# Autodesk Inventor assembly: Baugruppe
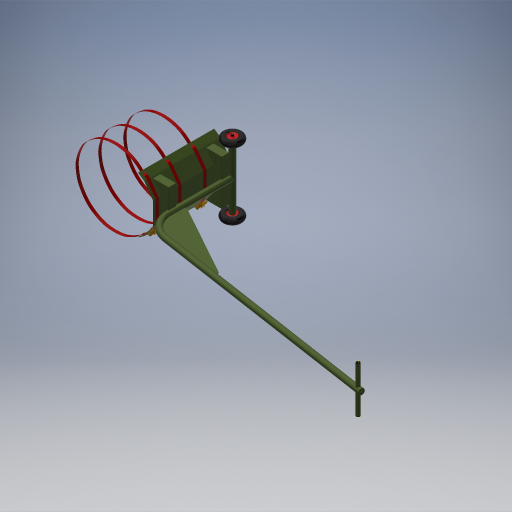
[picture p0: Inventor's stored thumbnail of the model, 512x512]
Saved by Autodesk Inventor 2023.2 (Build 272271000, 271)
## iProperties
Created: 2023-02-05
Part Number: Baugruppe
Material: Generisch
Document SubType Name: Assembly
Designer: Raoul Messerli
Author: Raoul Messerli
## Documents named in this file (8)
- E:\GitHub\Pflanzenwagen\40_Realisieren\20_Inventor\40_Baugruppen\Baugruppe.iam
- E:\GitHub\Pflanzenwagen\40_Realisieren\20_Inventor\40_Baugruppen\Schweiss Baugruppe.iam
- E:\GitHub\Pflanzenwagen\40_Realisieren\20_Inventor\20_Einkaufteile\Wheel.ipt
- E:\GitHub\Pflanzenwagen\40_Realisieren\20_Inventor\20_Einkaufteile\BN 161 1118811 prevailing torque type hex lock nut M20_Steel 6.ipt
- E:\GitHub\Pflanzenwagen\40_Realisieren\20_Inventor\20_Einkaufteile\Round_sliders.ipt
- E:\GitHub\Pflanzenwagen\40_Realisieren\20_Inventor\20_Einkaufteile\RatchetStrap\Strap for Pflanzenwagen.ipt
- E:\GitHub\Pflanzenwagen\40_Realisieren\20_Inventor\20_Einkaufteile\Gummi Matte.ipt
- E:\GitHub\Pflanzenwagen\40_Realisieren\20_Inventor\20_Einkaufteile\RatchetStrap\RatchetStrap\RatchetStrap.iam
## Components (14 placed, 7 different names)
1. Schweiss Baugruppe:1 [sub-assembly] — Fluchtend:1, Fluchtend:2, Fluchtend:3, Passend:1, Passend:2, Passend:3, Passend:4, Passend:5, Passend:7, Passend:9, Passend:10, Passend:11, Passend:12, Passend:14, Passend:18, Passend:21, Passend:22, Fluchtend:4, Passend:24, Passend:26, Passend:27
2. Wheel:1 — Passend:1, Passend:3, Passend:6
3. Wheel:2 — Passend:2, Passend:4, Passend:8
4. BN 161 1118811 prevailing torque type hex lock nut M20_Steel 6:1 — Passend:5, Passend:6
5. BN 161 1118811 prevailing torque type hex lock nut M20_Steel 6:2 — Passend:7, Passend:8
6. Round_sliders:1 — Passend:9, Passend:10
7. Round_sliders:2 — Passend:11, Passend:12
8. Strap for Pflanzenwagen:1 — Passend:13, Passend:14, Passend:15, Passend:29
9. Strap for Pflanzenwagen:2 — Passend:16, Passend:17, Passend:18, Passend:28
10. Strap for Pflanzenwagen:3 — Passend:19, Passend:20, Passend:21, Passend:25
11. Gummi Matte:1 — Passend:22, Fluchtend:4, Passend:23
12. RatchetStrap:1 [sub-assembly] — Passend:24, Passend:25
13. RatchetStrap:2 [sub-assembly] — Passend:26, Passend:28
14. RatchetStrap:3 [sub-assembly] — Passend:27, Passend:29
## Relationships (33: Mate 29, Flush 4)
- Fluchtend:1 [Flush]: Schweiss Baugruppe:1
- Fluchtend:2 [Flush]: Schweiss Baugruppe:1
- Fluchtend:3 [Flush]: Schweiss Baugruppe:1
- Passend:1 [Mate]: Schweiss Baugruppe:1 ↔ Wheel:1
- Passend:2 [Mate]: Schweiss Baugruppe:1 ↔ Wheel:2
- Passend:3 [Mate]: Schweiss Baugruppe:1 ↔ Wheel:1
- Passend:4 [Mate]: Schweiss Baugruppe:1 ↔ Wheel:2
- Passend:5 [Mate]: Schweiss Baugruppe:1 ↔ BN 161 1118811 prevailing torque type hex lock nut M20_Steel 6:1
- Passend:6 [Mate]: Wheel:1 ↔ BN 161 1118811 prevailing torque type hex lock nut M20_Steel 6:1
- Passend:7 [Mate]: Schweiss Baugruppe:1 ↔ BN 161 1118811 prevailing torque type hex lock nut M20_Steel 6:2
- Passend:8 [Mate]: Wheel:2 ↔ BN 161 1118811 prevailing torque type hex lock nut M20_Steel 6:2
- Passend:9 [Mate]: Schweiss Baugruppe:1 ↔ Round_sliders:1
- Passend:10 [Mate]: Schweiss Baugruppe:1 ↔ Round_sliders:1
- Passend:11 [Mate]: Schweiss Baugruppe:1 ↔ Round_sliders:2
- Passend:12 [Mate]: Schweiss Baugruppe:1 ↔ Round_sliders:2
- Passend:13 [Mate] (-1000 mm): Strap for Pflanzenwagen:1
- Passend:14 [Mate]: Schweiss Baugruppe:1 ↔ Strap for Pflanzenwagen:1
- Passend:15 [Mate] (-543 mm): Strap for Pflanzenwagen:1
- Passend:16 [Mate] (-1000 mm): Strap for Pflanzenwagen:2
- Passend:17 [Mate] (-543 mm): Strap for Pflanzenwagen:2
- Passend:18 [Mate]: Schweiss Baugruppe:1 ↔ Strap for Pflanzenwagen:2
- Passend:19 [Mate] (-1000 mm): Strap for Pflanzenwagen:3
- Passend:20 [Mate] (-543 mm): Strap for Pflanzenwagen:3
- Passend:21 [Mate]: Schweiss Baugruppe:1 ↔ Strap for Pflanzenwagen:3
- Passend:22 [Mate]: Schweiss Baugruppe:1 ↔ Gummi Matte:1
- Fluchtend:4 [Flush] (50 mm): Schweiss Baugruppe:1 ↔ Gummi Matte:1
- Passend:23 [Mate]: Gummi Matte:1
- Passend:24 [Mate]: Schweiss Baugruppe:1 ↔ RatchetStrap:1
- Passend:25 [Mate]: Strap for Pflanzenwagen:3 ↔ RatchetStrap:1
- Passend:26 [Mate]: Schweiss Baugruppe:1 ↔ RatchetStrap:2
- Passend:27 [Mate]: Schweiss Baugruppe:1 ↔ RatchetStrap:3
- Passend:28 [Mate]: Strap for Pflanzenwagen:2 ↔ RatchetStrap:2
- Passend:29 [Mate]: Strap for Pflanzenwagen:1 ↔ RatchetStrap:3
